# Autodesk Inventor assembly: Final
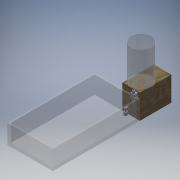
[picture p0: Inventor's stored thumbnail of the model, 180x180]
Saved by Autodesk Inventor 2018 (Build 220112000, 112)
## iProperties
Created: 2019-07-25
Part Number: Final
Document SubType Name: Assembly
Designer: micha
Author: micha
## Documents named in this file (8)
- C:\Users\micha\Documents\Inventor\Plants\Final.iam
- C:\Users\micha\Documents\Inventor\Plants\Breadboard.ipt
- C:\Users\micha\Documents\Inventor\Plants\Electronics_Box.ipt
- C:\Users\micha\Documents\Inventor\Plants\ESP8266 v7.iam
- C:\Users\micha\Documents\Inventor\Plants\Float_Switch.ipt
- C:\Users\micha\Documents\Inventor\Plants\PlantBox.ipt
- C:\Users\micha\Documents\Inventor\Plants\Valve.ipt
- C:\Users\micha\Documents\Inventor\Plants\Water Jug.ipt
## Components (7 placed, 7 different names)
1. Breadboard:1 — Mate:10, Mate:11, Mate:12, Mate:13, Mate:14, Mate:15
2. Electronics_Box:1 — Mate:1, Mate:2, Flush:1, Mate:3, Flush:2, Mate:4, Mate:9, Mate:10, Mate:11, Mate:12
3. ESP8266 v7:1 [sub-assembly] — Mate:13, Mate:14, Mate:15
4. Float_Switch:1 — Flush:3, Mate:7, Mate:8
5. PlantBox:1 — Mate:1, Mate:2, Flush:1, Mate:5, Mate:6, Flush:3, Mate:7, Mate:8
6. Valve:1 — Mate:4, Mate:5, Mate:6
7. Water Jug:1 — Mate:3, Flush:2, Mate:9
## Relationships (18: Mate 15, Flush 3)
- Mate:1: Electronics_Box:1 ↔ PlantBox:1
- Mate:2: Electronics_Box:1 ↔ PlantBox:1
- Flush:1: Electronics_Box:1 ↔ PlantBox:1
- Mate:3: Electronics_Box:1 ↔ Water Jug:1
- Flush:2: Electronics_Box:1 ↔ Water Jug:1
- Mate:4: Electronics_Box:1 ↔ Valve:1
- Mate:5: PlantBox:1 ↔ Valve:1
- Mate:6: PlantBox:1 ↔ Valve:1
- Flush:3 (76.2 mm): Float_Switch:1 ↔ PlantBox:1
- Mate:7: Float_Switch:1 ↔ PlantBox:1
- Mate:8 (50.8 mm): Float_Switch:1 ↔ PlantBox:1
- Mate:9 (-63.5 mm): Electronics_Box:1 ↔ Water Jug:1
- Mate:10: Breadboard:1 ↔ Electronics_Box:1
- Mate:11: Breadboard:1 ↔ Electronics_Box:1
- Mate:12: Breadboard:1 ↔ Electronics_Box:1
- Mate:13: Breadboard:1 ↔ ESP8266 v7:1
- Mate:14: Breadboard:1 ↔ ESP8266 v7:1
- Mate:15: Breadboard:1 ↔ ESP8266 v7:1
